# Autodesk Inventor assembly: 4-bar intake assebly 3
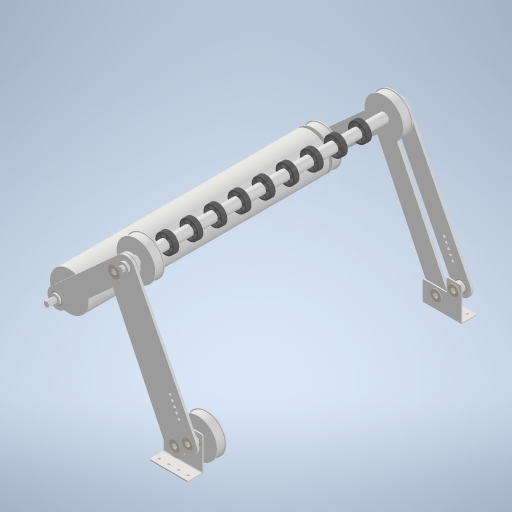
[picture p0: Inventor's stored thumbnail of the model, 512x512]
Saved by Autodesk Inventor 2023 (Build 270158030, 158C)
## iProperties
Created: 2022-07-21
Part Number: 4-bar intake assebly 3
Document SubType Name: Assembly
Designer: rm0990889
Author: rm0990889
## Documents named in this file (14)
- C:\Users\rm0990889\Downloads\4-bar intake assebly 3.iam
- C:\Users\rm0990889\Downloads\FIRST CAD-20220722T135427Z-001\FIRST CAD\4-bar intake practice-20220720T134858Z-001\4-bar intake practice\4-bar intake mount(alt).ipt
- C:\Users\rm0990889\Downloads\FIRST CAD-20220722T135427Z-001\FIRST CAD\4-bar intake practice-20220720T134858Z-001\4-bar intake practice\4-bar intake mount.ipt
- C:\Users\rm0990889\Downloads\FIRST CAD-20220722T135427Z-001\FIRST CAD\4-bar intake practice-20220720T134858Z-001\4-bar intake practice\am-2986 FR8ZZ Hex Bearing.ipt
- C:\Users\rm0990889\Downloads\FIRST CAD-20220722T135427Z-001\FIRST CAD\4-bar intake practice-20220720T134858Z-001\4-bar intake practice\4-bar intake (14.112) bar.ipt
- C:\Users\rm0990889\Downloads\FIRST CAD-20220722T135427Z-001\FIRST CAD\4-bar intake practice-20220720T134858Z-001\4-bar intake practice\4-bar intake (14.258) bar.ipt
- C:\Users\rm0990889\Downloads\FIRST CAD-20220722T135427Z-001\FIRST CAD\4-bar intake practice-20220720T134858Z-001\4-bar intake practice\4-bar intake block.ipt
- C:\Users\rm0990889\Downloads\FIRST CAD-20220722T135427Z-001\FIRST CAD\4-bar intake practice-20220720T134858Z-001\4-bar intake practice\4-bar intake spacer.ipt
- C:\Users\rm0990889\Downloads\FIRST CAD-20220722T135427Z-001\FIRST CAD\4-bar intake practice-20220720T134858Z-001\4-bar intake practice\4-bar intake shaft (29.5).ipt
- C:\Users\rm0990889\Downloads\FIRST CAD-20220722T135427Z-001\FIRST CAD\4-bar intake practice-20220720T134858Z-001\4-bar intake practice\4-bar intake () pully.ipt
- C:\Users\rm0990889\Downloads\FIRST CAD-20220722T135427Z-001\FIRST CAD\4-bar intake practice-20220720T134858Z-001\4-bar intake practice\4-bar intake (1_) spacer.ipt
- C:\Users\rm0990889\Downloads\FIRST CAD-20220722T135427Z-001\FIRST CAD\4-bar intake practice-20220720T134858Z-001\4-bar intake practice\4-bar intake (2_) spacer.ipt
- C:\Users\rm0990889\Downloads\FIRST CAD-20220722T135427Z-001\FIRST CAD\4-bar intake practice-20220720T134858Z-001\4-bar intake practice\am-3462 2IN Molded 500Hex Compliant Wheel REV2.ipt
- C:\Users\rm0990889\Downloads\FIRST CAD-20220722T135427Z-001\FIRST CAD\4-bar intake practice-20220720T134858Z-001\4-bar intake practice\4-bar intake roller (25).ipt
## Components (67 placed, 13 different names)
1. 4-bar intake mount(alt):1 — Flush:1, Flush:2, Mate:1, Insert:1, Insert:2
2. 4-bar intake mount:1 — Flush:1, Flush:2, Mate:1, Insert:3, Insert:4
3. am-2986 FR8ZZ Hex Bearing:1 — Insert:3, Insert:23, Flush:7, Insert:29
4. am-2986 FR8ZZ Hex Bearing:2 — Insert:8, Mate:2, Flush:5
5. am-2986 FR8ZZ Hex Bearing:3 — Insert:7, Insert:19, Flush:8
6. am-2986 FR8ZZ Hex Bearing:4 — Insert:4, Insert:19, Flush:8
7. am-2986 FR8ZZ Hex Bearing:5 — Insert:1, Insert:21
8. am-2986 FR8ZZ Hex Bearing:6 — Insert:2, Insert:20
9. am-2986 FR8ZZ Hex Bearing:7 — Insert:6, Insert:25
10. am-2986 FR8ZZ Hex Bearing:8 — Insert:5, Flush:6, Insert:62
11. 4-bar intake (14.112) bar:1 — Insert:7, Insert:8
12. 4-bar intake (14.112) bar:2 — Insert:14, Insert:15
13. 4-bar intake (14.258) bar:1 — Insert:5, Insert:6, Insert:27
14. 4-bar intake (14.258) bar:2 — Insert:12, Insert:13, Insert:60
15. 4-bar intake block:1 — Insert:16, Insert:17, Insert:18, Insert:56
16. 4-bar intake block:2 — Insert:9, Insert:10, Insert:11
17. am-2986 FR8ZZ Hex Bearing:9 — Insert:9, Insert:27, Flush:6, Mate:10, Mate:11, Insert:30
18. am-2986 FR8ZZ Hex Bearing:10 — Insert:10, Mate:2, Flush:5
19. am-2986 FR8ZZ Hex Bearing:11 — Insert:11, Mate:6, Mate:7, Insert:33, Insert:63
20. am-2986 FR8ZZ Hex Bearing:12 — Insert:12, Insert:28, Flush:3, Mate:8, Mate:9
21. am-2986 FR8ZZ Hex Bearing:13 — Insert:13, Insert:26
22. am-2986 FR8ZZ Hex Bearing:14 — Insert:14, Insert:20
23. am-2986 FR8ZZ Hex Bearing:15 — Insert:15, Mate:3, Flush:4
24. am-2986 FR8ZZ Hex Bearing:16 — Insert:16, Insert:28, Flush:3
25. am-2986 FR8ZZ Hex Bearing:17 — Insert:17, Mate:3, Flush:4
26. am-2986 FR8ZZ Hex Bearing:18 — Insert:18, Mate:4, Mate:5, Insert:61
27. 4-bar intake spacer:1 — Insert:23, Insert:24, Flush:7
28. 4-bar intake spacer:2 — Insert:24, Insert:25
29. 4-bar intake spacer:3 — Insert:22, Insert:26
30. 4-bar intake spacer:4 — Insert:21, Insert:22
31. 4-bar intake shaft (29.5):1 — Mate:4, Mate:5, Mate:6, Mate:7, Flush:10
32. 4-bar intake shaft (29.5):2 — Mate:8, Mate:9, Mate:10, Mate:11, Flush:9
33. 4-bar intake () pully:1 — Insert:29
34. 4-bar intake () pully:2 — Insert:32, Insert:34
35. 4-bar intake () pully:3 — Insert:54, Insert:55
36. 4-bar intake () pully:4 — Insert:57, Insert:59
37. 4-bar intake spacer:5 — Insert:30, Insert:31
38. 4-bar intake spacer:6 — Insert:56, Insert:57
39. 4-bar intake spacer:7 — Insert:31, Insert:32
40. 4-bar intake spacer:8 — Insert:62
41. 4-bar intake spacer:9 — Insert:55
42. 4-bar intake spacer:10 — Insert:59
43. 4-bar intake spacer:12 — Insert:53, Insert:54
44. 4-bar intake (1_) spacer:1 — Insert:33, Insert:58
45. 4-bar intake (2_) spacer:3 — Insert:42, Insert:43
46. 4-bar intake (2_) spacer:4 — Insert:38, Insert:39
47. 4-bar intake (2_) spacer:5 — Insert:36, Insert:37
48. 4-bar intake (2_) spacer:6 — Insert:40, Insert:41
49. 4-bar intake (2_) spacer:7 — Insert:34, Insert:35
50. 4-bar intake (2_) spacer:8 — Insert:46, Insert:47
51. 4-bar intake (2_) spacer:9 — Insert:48, Insert:49
52. 4-bar intake (2_) spacer:10 — Insert:50, Insert:51
53. 4-bar intake (2_) spacer:11 — Insert:52, Insert:53
54. 4-bar intake (2_) spacer:12 — Insert:44, Insert:45
55. am-3462 2IN Molded 500Hex Compliant Wheel REV2:1 — Insert:41, Insert:42
56. am-3462 2IN Molded 500Hex Compliant Wheel REV2:2 — Insert:39, Insert:40
57. am-3462 2IN Molded 500Hex Compliant Wheel REV2:3 — Insert:35, Insert:36
58. am-3462 2IN Molded 500Hex Compliant Wheel REV2:4 — Insert:37, Insert:38
59. am-3462 2IN Molded 500Hex Compliant Wheel REV2:5 — Insert:47, Insert:48
60. am-3462 2IN Molded 500Hex Compliant Wheel REV2:6 — Insert:45, Insert:46
61. am-3462 2IN Molded 500Hex Compliant Wheel REV2:7 — Insert:49, Insert:50
62. am-3462 2IN Molded 500Hex Compliant Wheel REV2:8 — Insert:51, Insert:52
63. am-3462 2IN Molded 500Hex Compliant Wheel REV2:12 — Insert:43, Insert:44
64. 4-bar intake roller (25):1 — Insert:58
65. 4-bar intake spacer:13 — Insert:60, Flush:9
66. 4-bar intake spacer:14 — Insert:61, Flush:10
67. 4-bar intake spacer:15 — Insert:63
## Relationships (84: Insert 63, Mate 11, Flush 10)
- Flush:1: 4-bar intake mount(alt):1 ↔ 4-bar intake mount:1
- Flush:2: 4-bar intake mount(alt):1 ↔ 4-bar intake mount:1
- Mate:1 (-762 mm): 4-bar intake mount(alt):1 ↔ 4-bar intake mount:1
- Insert:1: 4-bar intake mount(alt):1 ↔ am-2986 FR8ZZ Hex Bearing:5
- Insert:2: 4-bar intake mount(alt):1 ↔ am-2986 FR8ZZ Hex Bearing:6
- Insert:3: 4-bar intake mount:1 ↔ am-2986 FR8ZZ Hex Bearing:1
- Insert:4: 4-bar intake mount:1 ↔ am-2986 FR8ZZ Hex Bearing:4
- Insert:5: am-2986 FR8ZZ Hex Bearing:8 ↔ 4-bar intake (14.258) bar:1
- Insert:6: am-2986 FR8ZZ Hex Bearing:7 ↔ 4-bar intake (14.258) bar:1
- Insert:7: am-2986 FR8ZZ Hex Bearing:3 ↔ 4-bar intake (14.112) bar:1
- Insert:8: am-2986 FR8ZZ Hex Bearing:2 ↔ 4-bar intake (14.112) bar:1
- Insert:9: 4-bar intake block:2 ↔ am-2986 FR8ZZ Hex Bearing:9
- Insert:10: 4-bar intake block:2 ↔ am-2986 FR8ZZ Hex Bearing:10
- Insert:11: 4-bar intake block:2 ↔ am-2986 FR8ZZ Hex Bearing:11
- Insert:12: 4-bar intake (14.258) bar:2 ↔ am-2986 FR8ZZ Hex Bearing:12
- Insert:13: 4-bar intake (14.258) bar:2 ↔ am-2986 FR8ZZ Hex Bearing:13
- Insert:14: 4-bar intake (14.112) bar:2 ↔ am-2986 FR8ZZ Hex Bearing:14
- Insert:15: 4-bar intake (14.112) bar:2 ↔ am-2986 FR8ZZ Hex Bearing:15
- Insert:16: 4-bar intake block:1 ↔ am-2986 FR8ZZ Hex Bearing:16
- Insert:17: 4-bar intake block:1 ↔ am-2986 FR8ZZ Hex Bearing:17
- Insert:18: 4-bar intake block:1 ↔ am-2986 FR8ZZ Hex Bearing:18
- Insert:19: am-2986 FR8ZZ Hex Bearing:3 ↔ am-2986 FR8ZZ Hex Bearing:4
- Insert:20: am-2986 FR8ZZ Hex Bearing:6 ↔ am-2986 FR8ZZ Hex Bearing:14
- Insert:21: am-2986 FR8ZZ Hex Bearing:5 ↔ 4-bar intake spacer:4
- Insert:22: 4-bar intake spacer:3 ↔ 4-bar intake spacer:4
- Insert:23: am-2986 FR8ZZ Hex Bearing:1 ↔ 4-bar intake spacer:1
- Insert:24: 4-bar intake spacer:1 ↔ 4-bar intake spacer:2
- Insert:25: am-2986 FR8ZZ Hex Bearing:7 ↔ 4-bar intake spacer:2
- Insert:26: am-2986 FR8ZZ Hex Bearing:13 ↔ 4-bar intake spacer:3
- Insert:27: 4-bar intake (14.258) bar:1 ↔ am-2986 FR8ZZ Hex Bearing:9
- Mate:2: am-2986 FR8ZZ Hex Bearing:2 ↔ am-2986 FR8ZZ Hex Bearing:10
- Insert:28: am-2986 FR8ZZ Hex Bearing:12 ↔ am-2986 FR8ZZ Hex Bearing:16
- Mate:3: am-2986 FR8ZZ Hex Bearing:15 ↔ am-2986 FR8ZZ Hex Bearing:17
- Mate:4: am-2986 FR8ZZ Hex Bearing:18 ↔ 4-bar intake shaft (29.5):1
- Mate:5: am-2986 FR8ZZ Hex Bearing:18 ↔ 4-bar intake shaft (29.5):1
- Flush:3: am-2986 FR8ZZ Hex Bearing:12 ↔ am-2986 FR8ZZ Hex Bearing:16
- Flush:4: am-2986 FR8ZZ Hex Bearing:15 ↔ am-2986 FR8ZZ Hex Bearing:17
- Flush:5: am-2986 FR8ZZ Hex Bearing:2 ↔ am-2986 FR8ZZ Hex Bearing:10
- Flush:6: am-2986 FR8ZZ Hex Bearing:8 ↔ am-2986 FR8ZZ Hex Bearing:9
- Flush:7: am-2986 FR8ZZ Hex Bearing:1 ↔ 4-bar intake spacer:1
- Flush:8: am-2986 FR8ZZ Hex Bearing:3 ↔ am-2986 FR8ZZ Hex Bearing:4
- Mate:6: am-2986 FR8ZZ Hex Bearing:11 ↔ 4-bar intake shaft (29.5):1
- Mate:7: am-2986 FR8ZZ Hex Bearing:11 ↔ 4-bar intake shaft (29.5):1
- Mate:8: am-2986 FR8ZZ Hex Bearing:12 ↔ 4-bar intake shaft (29.5):2
- Mate:9: am-2986 FR8ZZ Hex Bearing:12 ↔ 4-bar intake shaft (29.5):2
- Mate:10: am-2986 FR8ZZ Hex Bearing:9 ↔ 4-bar intake shaft (29.5):2
- Mate:11: am-2986 FR8ZZ Hex Bearing:9 ↔ 4-bar intake shaft (29.5):2
- Insert:29: am-2986 FR8ZZ Hex Bearing:1 ↔ 4-bar intake () pully:1
- Insert:30: am-2986 FR8ZZ Hex Bearing:9 ↔ 4-bar intake spacer:5
- Insert:31: 4-bar intake spacer:5 ↔ 4-bar intake spacer:7
- Insert:32: 4-bar intake () pully:2 ↔ 4-bar intake spacer:7
- Insert:33: am-2986 FR8ZZ Hex Bearing:11 ↔ 4-bar intake (1_) spacer:1
- Insert:34: 4-bar intake () pully:2 ↔ 4-bar intake (2_) spacer:7
- Insert:35: 4-bar intake (2_) spacer:7 ↔ am-3462 2IN Molded 500Hex Compliant Wheel REV2:3
- Insert:36: 4-bar intake (2_) spacer:5 ↔ am-3462 2IN Molded 500Hex Compliant Wheel REV2:3
- Insert:37: 4-bar intake (2_) spacer:5 ↔ am-3462 2IN Molded 500Hex Compliant Wheel REV2:4
- Insert:38: 4-bar intake (2_) spacer:4 ↔ am-3462 2IN Molded 500Hex Compliant Wheel REV2:4
- Insert:39: 4-bar intake (2_) spacer:4 ↔ am-3462 2IN Molded 500Hex Compliant Wheel REV2:2
- Insert:40: 4-bar intake (2_) spacer:6 ↔ am-3462 2IN Molded 500Hex Compliant Wheel REV2:2
- Insert:41: 4-bar intake (2_) spacer:6 ↔ am-3462 2IN Molded 500Hex Compliant Wheel REV2:1
- Insert:42: 4-bar intake (2_) spacer:3 ↔ am-3462 2IN Molded 500Hex Compliant Wheel REV2:1
- Insert:43: 4-bar intake (2_) spacer:3 ↔ am-3462 2IN Molded 500Hex Compliant Wheel REV2:12
- Insert:44: 4-bar intake (2_) spacer:12 ↔ am-3462 2IN Molded 500Hex Compliant Wheel REV2:12
- Insert:45: 4-bar intake (2_) spacer:12 ↔ am-3462 2IN Molded 500Hex Compliant Wheel REV2:6
- Insert:46: 4-bar intake (2_) spacer:8 ↔ am-3462 2IN Molded 500Hex Compliant Wheel REV2:6
- Insert:47: 4-bar intake (2_) spacer:8 ↔ am-3462 2IN Molded 500Hex Compliant Wheel REV2:5
- Insert:48: 4-bar intake (2_) spacer:9 ↔ am-3462 2IN Molded 500Hex Compliant Wheel REV2:5
- Insert:49: 4-bar intake (2_) spacer:9 ↔ am-3462 2IN Molded 500Hex Compliant Wheel REV2:7
- Insert:50: 4-bar intake (2_) spacer:10 ↔ am-3462 2IN Molded 500Hex Compliant Wheel REV2:7
- Insert:51: 4-bar intake (2_) spacer:10 ↔ am-3462 2IN Molded 500Hex Compliant Wheel REV2:8
- Insert:52: 4-bar intake (2_) spacer:11 ↔ am-3462 2IN Molded 500Hex Compliant Wheel REV2:8
- Insert:53: 4-bar intake spacer:12 ↔ 4-bar intake (2_) spacer:11
- Insert:54: 4-bar intake () pully:3 ↔ 4-bar intake spacer:12
- Insert:55: 4-bar intake () pully:3 ↔ 4-bar intake spacer:9
- Insert:56: 4-bar intake block:1 ↔ 4-bar intake spacer:6
- Insert:57: 4-bar intake () pully:4 ↔ 4-bar intake spacer:6
- Insert:58: 4-bar intake (1_) spacer:1 ↔ 4-bar intake roller (25):1
- Insert:59: 4-bar intake () pully:4 ↔ 4-bar intake spacer:10
- Insert:60: 4-bar intake (14.258) bar:2 ↔ 4-bar intake spacer:13
- Flush:9: 4-bar intake shaft (29.5):2 ↔ 4-bar intake spacer:13
- Insert:61: am-2986 FR8ZZ Hex Bearing:18 ↔ 4-bar intake spacer:14
- Flush:10: 4-bar intake shaft (29.5):1 ↔ 4-bar intake spacer:14
- Insert:62: am-2986 FR8ZZ Hex Bearing:8 ↔ 4-bar intake spacer:8
- Insert:63: am-2986 FR8ZZ Hex Bearing:11 ↔ 4-bar intake spacer:15
